# Autodesk Inventor assembly: Hinge 5 Holes_CPY
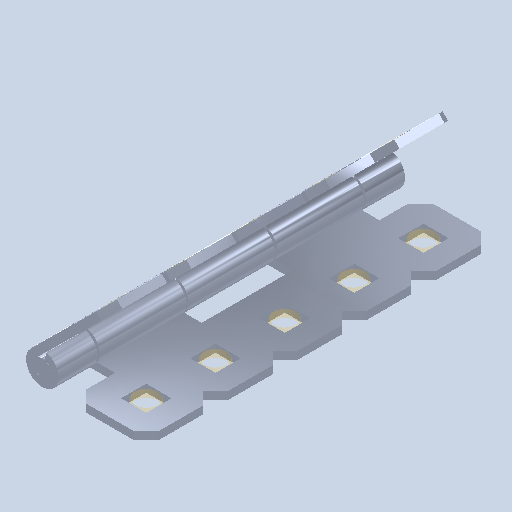
[picture p0: Inventor's stored thumbnail of the model, 512x512]
Saved by Autodesk Inventor 2022 (Build 260153070, 153G)
## iProperties
Category: Structure
Company: Super Sonic Sparks, Team 24
Created: 2019-06-17
Part Number: Hinge 5 Holes_CPY
Catalog Web Link: vexrobotics.com/275-1272.html
Description: Provides a simple pivoting joint.
Vendor: VEX Robotics, Inc.
Document SubType Name: Assembly
Designer: Main Account
Mass: 29.4658 g
Surface Area: 66.2962 cm^2
Volume: 4.04593 cm^3
Density: 7.28282 g/cm^3
Title: Hinge
Author: Jordan Kiesel
Comments: This hinge provides a simple pivoting joint with 265 degree movement. ▷ 2.5" long x 1.3" wide. ▷ Standard VEX holes.
Translation Standard: STEP AP203
FileName: Hinge.iam
PreProcessor: SolidWorks 2010
PostProcessor: Build: 160, Release: 2012 RTM - Date: Tue 03/01/2011
Sent Units: inch
Uncertainty: 1e-05
## Documents named in this file (4)
- D:\Documents\Inventor\VEX\Projects\ChangeUpFinal\Library\Library 1.2\Mirror Dump\Hinge 5 Holes_CPY.iam
- D:\Documents\Inventor\VEX\Projects\ChangeUpFinal\Library\Library 1.2\Mirror Dump\Bottom 5_CPY.ipt
- D:\Documents\Inventor\VEX\Projects\ChangeUpFinal\Library\Library 1.2\Mirror Dump\Pin 5_CPY.ipt
- D:\Documents\Inventor\VEX\Projects\ChangeUpFinal\Library\Library 1.2\Mirror Dump\Top 5_CPY.ipt
## Components (3 placed, 3 different names)
1. Bottom 5_CPY:1 — Mate:3, Mate:2
2. Pin 5_CPY:1 — Mate:1, Flush:1, Mate:3
3. Top 5_CPY:1 — Mate:1, Flush:1, Mate:2
## Relationships (4: Mate 3, Flush 1)
- Mate:1: Pin 5_CPY:1 ↔ Top 5_CPY:1
- Flush:1: Pin 5_CPY:1 ↔ Top 5_CPY:1
- Mate:3: Bottom 5_CPY:1 ↔ Pin 5_CPY:1
- Mate:2 (0.4064 mm): Bottom 5_CPY:1 ↔ Top 5_CPY:1
